# Autodesk Inventor assembly: 005
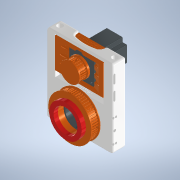
[picture p0: Inventor's stored thumbnail of the model, 180x180]
Saved by Autodesk Inventor 2020 (Build 240168000, 168)
## iProperties
Created: 2024-06-19
Part Number: 005
Document SubType Name: Assembly
Designer: Scott Bricker
Project: Motorized Rotator Mount
Description: Motorized Rotator Mount Assembly
Engineer: Scott Bricker
Author: Scott Bricker
Title: Motorized Rotator Mount Assembly
Revision Number: v1.0
## Documents named in this file (8)
- C:\Users\Scott\Documents\Inventor\THz Rotator Mount\v2.2a\Models\Motorized Rotator Mount Assembly.iam
- C:\Users\Scott\Documents\Inventor\THz Rotator Mount\Rotator Mount Base v2.2.ipt
- C:\Users\Scott\Documents\Inventor\THz Rotator Mount\Optical Mount.ipt
- C:\Users\Scott\Documents\Inventor\THz Rotator Mount\Stepper Motor Housing v2.2.ipt
- C:\Users\Scott\Documents\Inventor\THz Rotator Mount\Stepper Motor.ipt
- C:\Users\Scott\Documents\Inventor\THz Rotator Mount\Output Gear Actuator.ipt
- C:\Users\Scott\Documents\Inventor\THz Rotator Mount\Motor Gear Attachment v2.2.ipt
- C:\Users\Scott\Documents\Inventor\THz Rotator Mount\THz Polarizer.ipt
## Components (7 placed, 7 different names)
1. Rotator Mount Base v2.2:1 — Mate:1, Mate:2, Mate:3, Mate:4, Mate:5
2. Optical Mount:1 — Mate:1, Mate:2, Mate:3, Insert:2
3. Stepper Motor Housing v2.2:1 — Mate:4, Mate:5, Mate:6, Mate:7, Mate:8
4. Stepper Motor:1 — Mate:6, Mate:7, Mate:8, Insert:1
5. Output Gear Actuator:1 — Insert:2, Insert:3, Insert:4
6. Motor Gear Attachment v2.2:1 — Insert:1
7. THz Polarizer:1 — Insert:3, Insert:4
## Relationships (12: Mate 8, Insert 4)
- Mate:1: Rotator Mount Base v2.2:1 ↔ Optical Mount:1
- Mate:2 (0.15 mm): Rotator Mount Base v2.2:1 ↔ Optical Mount:1
- Mate:3 (0.15 mm): Rotator Mount Base v2.2:1 ↔ Optical Mount:1
- Mate:4 (0.5 mm): Rotator Mount Base v2.2:1 ↔ Stepper Motor Housing v2.2:1
- Mate:5: Rotator Mount Base v2.2:1 ↔ Stepper Motor Housing v2.2:1
- Mate:6: Stepper Motor Housing v2.2:1 ↔ Stepper Motor:1
- Mate:7: Stepper Motor Housing v2.2:1 ↔ Stepper Motor:1
- Mate:8: Stepper Motor Housing v2.2:1 ↔ Stepper Motor:1
- Insert:1 (4.9 mm): Stepper Motor:1 ↔ Motor Gear Attachment v2.2:1
- Insert:2: Optical Mount:1 ↔ Output Gear Actuator:1
- Insert:3: Output Gear Actuator:1 ↔ THz Polarizer:1
- Insert:4: Output Gear Actuator:1 ↔ THz Polarizer:1
